# Autodesk Inventor assembly: X Rail assy
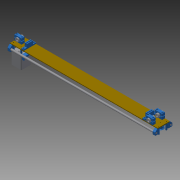
[picture p0: Inventor's stored thumbnail of the model, 180x180]
Saved by Autodesk Inventor 2013 SP2 (Build 170200200, 200)
## iProperties
Created: 2017-01-25
Part Number: X Rail assy
Document SubType Name: Assembly
Designer: Herman de Vries
Author: Herman de Vries
## Documents named in this file (14)
- E:\_hdv\Projects\PainterBot\X Rail assy.iam
- E:\_hdv\Projects\PainterBot\X Rail.ipt
- E:\_hdv\Projects\PainterBot\NEMA42.ipt
- E:\_hdv\Projects\PainterBot\gear belt.ipt
- E:\_hdv\Projects\PainterBot\switch lever.ipt
- E:\_hdv\Projects\PainterBot\Pully25mmx12mm.iam
- E:\_hdv\Projects\PainterBot\spacer 6mmx10_5mm.ipt
- E:\_hdv\Projects\PainterBot\spacer top 6mm.ipt
- E:\_hdv\Projects\PainterBot\spacer stepperM.ipt
- E:\_hdv\Projects\PainterBot\spacer stepperM n rail.ipt
- E:\_hdv\Projects\PainterBot\x axis 8mm rod.ipt
- E:\_hdv\Projects\PainterBot\8mm Rod clamp.ipt
- E:\_hdv\Projects\PainterBot\Linear bearing 8mm.ipt
- E:\_hdv\Projects\PainterBot\GT2 grip.ipt
## Components (24 placed, 13 different names)
1. X Rail:1 — Insert:4, Mate:1, Mate:11, Mate:14, Insert:26, Insert:27, Insert:28, Insert:29, Flush:14, Mate:17, Mate:18, Mate:19, Flush:15, Flush:16, Flush:17, Flush:18, Mate:21, Flush:21, Flush:22, Mate:22, Flush:23, Flush:24, Insert:33
2. NEMA42:1 — Insert:4, Mate:1, Mate:8, Mate:9, Mate:20
3. gear belt:1 — Mate:20
4. Pully25mmx12mm:1 [sub-assembly] — Insert:19, Insert:20
5. switch lever:1 — Mate:8, Mate:9
6. spacer 6mmx10_5mm:1 — Insert:19, Insert:33
7. spacer top 6mm:1 — Insert:20
8. spacer stepperM:2 — Insert:27
9. spacer stepperM:3 — Insert:26
10. spacer stepperM n rail:1 — Mate:11, Mate:15, Insert:28, Insert:29
11. spacer stepperM n rail:2 — Mate:14, Mate:15, Insert:24, Insert:25, Flush:14
12. x axis 8mm rod:1 — Insert:24
13. x axis 8mm rod:2 — Insert:25
14. 8mm Rod clamp:1 — Mate:17, Flush:15, Flush:16, Insert:30, Flush:20, Mate:24
15. 8mm Rod clamp:2 — Mate:18, Insert:31, Flush:18, Flush:19, Flush:20, Mate:28
16. 8mm Rod clamp:4 — Mate:19, Insert:32, Flush:17, Flush:19, Mate:27
17. Linear bearing 8mm:1 — Insert:30, Mate:23
18. Linear bearing 8mm:2 — Insert:31, Mate:25
19. Linear bearing 8mm:3 — Insert:32, Mate:26
20. GT2 grip:1 — Mate:21, Flush:21, Flush:22
21. GT2 grip:2 — Mate:22, Flush:23, Flush:24
22. 8mm Rod clamp:5 — Mate:23, Mate:24
23. 8mm Rod clamp:6 — Mate:26, Mate:27
24. 8mm Rod clamp:7 — Mate:25, Mate:28
## Relationships (42: Mate 18, Insert 13, Flush 11)
- Insert:4 (26 mm): X Rail:1 ↔ NEMA42:1
- Mate:1: X Rail:1 ↔ NEMA42:1
- Mate:8: NEMA42:1 ↔ switch lever:1
- Mate:9: NEMA42:1 ↔ switch lever:1
- Insert:19: Pully25mmx12mm:1 ↔ spacer 6mmx10_5mm:1
- Insert:20: Pully25mmx12mm:1 ↔ spacer top 6mm:1
- Mate:11: X Rail:1 ↔ spacer stepperM n rail:1
- Mate:14: X Rail:1 ↔ spacer stepperM n rail:2
- Mate:15: spacer stepperM n rail:1 ↔ spacer stepperM n rail:2
- Insert:24: spacer stepperM n rail:2 ↔ x axis 8mm rod:1
- Insert:25: spacer stepperM n rail:2 ↔ x axis 8mm rod:2
- Insert:26: X Rail:1 ↔ spacer stepperM:3
- Insert:27: X Rail:1 ↔ spacer stepperM:2
- Insert:28: X Rail:1 ↔ spacer stepperM n rail:1
- Insert:29: X Rail:1 ↔ spacer stepperM n rail:1
- Flush:14: X Rail:1 ↔ spacer stepperM n rail:2
- Mate:17: X Rail:1 ↔ 8mm Rod clamp:1
- Mate:18: X Rail:1 ↔ 8mm Rod clamp:2
- Mate:19: X Rail:1 ↔ 8mm Rod clamp:4
- Flush:15: X Rail:1 ↔ 8mm Rod clamp:1
- Flush:16 (-17.5 mm): X Rail:1 ↔ 8mm Rod clamp:1
- Insert:30 (-5 mm): 8mm Rod clamp:1 ↔ Linear bearing 8mm:1
- Insert:31 (-5 mm): 8mm Rod clamp:2 ↔ Linear bearing 8mm:2
- Insert:32 (-5 mm): 8mm Rod clamp:4 ↔ Linear bearing 8mm:3
- Flush:17: X Rail:1 ↔ 8mm Rod clamp:4
- Flush:18: X Rail:1 ↔ 8mm Rod clamp:2
- Flush:19: 8mm Rod clamp:2 ↔ 8mm Rod clamp:4
- Flush:20 (560 mm): 8mm Rod clamp:1 ↔ 8mm Rod clamp:2
- Mate:20: NEMA42:1 ↔ gear belt:1
- Mate:21: X Rail:1 ↔ GT2 grip:1
- Flush:21: X Rail:1 ↔ GT2 grip:1
- Flush:22 (47 mm): X Rail:1 ↔ GT2 grip:1
- Mate:22: X Rail:1 ↔ GT2 grip:2
- Flush:23: X Rail:1 ↔ GT2 grip:2
- Flush:24 (-53 mm): X Rail:1 ↔ GT2 grip:2
- Insert:33: X Rail:1 ↔ spacer 6mmx10_5mm:1
- Mate:23: Linear bearing 8mm:1 ↔ 8mm Rod clamp:5
- Mate:24: 8mm Rod clamp:1 ↔ 8mm Rod clamp:5
- Mate:25: Linear bearing 8mm:2 ↔ 8mm Rod clamp:7
- Mate:26: Linear bearing 8mm:3 ↔ 8mm Rod clamp:6
- Mate:27: 8mm Rod clamp:4 ↔ 8mm Rod clamp:6
- Mate:28: 8mm Rod clamp:2 ↔ 8mm Rod clamp:7
